# Autodesk Inventor assembly: ASY МОО 020 конус
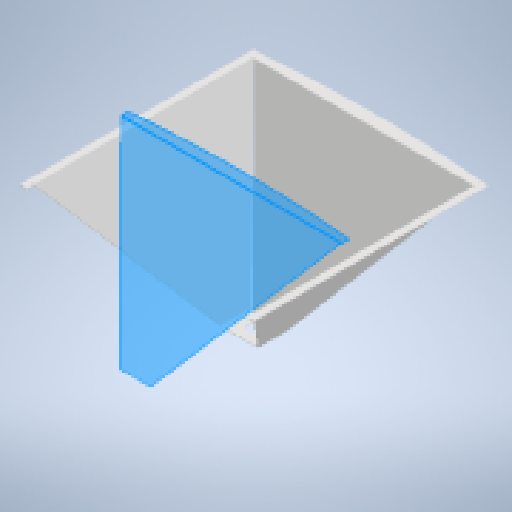
[picture p0: Inventor's stored thumbnail of the model, 512x512]
Saved by Autodesk Inventor 2024.2 (Build 282272000, 272)
## iProperties
Created: 2024-05-19
Part Number: ASY МОО 020 конус
Document SubType Name: Assembly
Designer: admin
Author: admin
## Documents named in this file (6)
- C:\Users\admin\YandexDisk-badmisterfox\домашниий пк\Inventor\Manturovo\отстойник осветлитель\ASY МОО 020 конус.iam
- C:\Users\admin\YandexDisk-badmisterfox\домашниий пк\Inventor\Manturovo\отстойник осветлитель\конус\МОО 023 конус правый борт 1.ipt
- C:\Users\admin\YandexDisk-badmisterfox\домашниий пк\Inventor\Manturovo\отстойник осветлитель\конус\МОО 029 конус дно.ipt
- C:\Users\admin\YandexDisk-badmisterfox\домашниий пк\Inventor\Manturovo\отстойник осветлитель\конус\МОО 025 конус левый борт 1.ipt
- C:\Users\admin\YandexDisk-badmisterfox\домашниий пк\Inventor\Manturovo\отстойник осветлитель\конус\МОО 022 конус корма.ipt
- C:\Users\admin\YandexDisk-badmisterfox\домашниий пк\Inventor\Manturovo\отстойник осветлитель\конус\МОО 026 конус корма.ipt
## Components (6 placed, 5 different names)
1. МОО 029 конус дно:1 — Flush:4, Flush:5
2. МОО 023 конус правый борт 1:1 — Flush:1, Rigid:2, Rigid:3, Rigid:4
3. МОО 025 конус левый борт 1:1 — Rigid:1
4. МОО 022 конус корма:1 — Flush:6, Flush:7, Rigid:1, Rigid:2
5. МОО 026 конус корма:1 — Mate:10, Rigid:3
6. МОО 023 конус правый борт 1:2 — Rigid:4
## Relationships (10: Flush 5, WeldJoint 4, Mate 1)
- Flush:1: МОО 023 конус правый борт 1:1
- Flush:4: МОО 029 конус дно:1
- Flush:5: МОО 029 конус дно:1
- Flush:6: МОО 022 конус корма:1
- Flush:7: МОО 022 конус корма:1
- Mate:10: МОО 026 конус корма:1
- Rigid:1 [WeldJoint]: МОО 025 конус левый борт 1:1 ↔ МОО 022 конус корма:1
- Rigid:2 [WeldJoint]: МОО 023 конус правый борт 1:1 ↔ МОО 022 конус корма:1
- Rigid:3 [WeldJoint]: МОО 023 конус правый борт 1:1 ↔ МОО 026 конус корма:1
- Rigid:4 [WeldJoint]: МОО 023 конус правый борт 1:1 ↔ МОО 023 конус правый борт 1:2
